# Autodesk Inventor assembly: HALF GANTRY ASSEMBLY
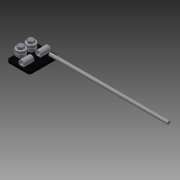
[picture p0: Inventor's stored thumbnail of the model, 180x180]
Saved by Autodesk Inventor 2013 (Build 170138000, 138)
## iProperties
Created: 2014-03-03
Part Number: HALF GANTRY ASSEMBLY
Document SubType Name: Assembly
Designer: employee
Author: employee
## Documents named in this file (8)
- C:\Users\employee\Desktop\CoreXZ\HALF GANTRY ASSEMBLY.iam
- C:\Users\employee\Desktop\CoreXZ\GANTRY SIDE PLATE.ipt
- C:\Users\employee\Desktop\CoreXZ\LM8UU.ipt
- C:\Users\employee\Desktop\CoreXZ\M8X290 ROD.ipt
- C:\Users\employee\Desktop\CoreXZ\SPACER.ipt
- C:\Users\employee\Desktop\CoreXZ\608.ipt
- C:\Users\employee\Desktop\CoreXZ\M8X40.ipt
- C:\Users\employee\Desktop\CoreXZ\M8 NUT.ipt
## Components (14 placed, 7 different names)
1. GANTRY SIDE PLATE:1 — Insert:1, Insert:2, Insert:3, Insert:4, Insert:5, Insert:12, Insert:13
2. LM8UU:1 — Insert:1
3. LM8UU:2 — Insert:2
4. M8X290 ROD:1 — Insert:3
5. SPACER:1 — Insert:5, Insert:8
6. SPACER:2 — Insert:4, Insert:6
7. 608:1 — Insert:7, Insert:10
8. 608:2 — Insert:6, Insert:7
9. 608:3 — Insert:8, Insert:9
10. 608:4 — Insert:9, Insert:11
11. M8X40:1 — Insert:10
12. M8X40:2 — Insert:11
13. M8 NUT:1 — Insert:12
14. M8 NUT:2 — Insert:13
## Relationships (13: Insert 13)
- Insert:1: GANTRY SIDE PLATE:1 ↔ LM8UU:1
- Insert:2: GANTRY SIDE PLATE:1 ↔ LM8UU:2
- Insert:3: GANTRY SIDE PLATE:1 ↔ M8X290 ROD:1
- Insert:4: GANTRY SIDE PLATE:1 ↔ SPACER:2
- Insert:5: GANTRY SIDE PLATE:1 ↔ SPACER:1
- Insert:6: SPACER:2 ↔ 608:2
- Insert:7: 608:1 ↔ 608:2
- Insert:8: SPACER:1 ↔ 608:3
- Insert:9: 608:3 ↔ 608:4
- Insert:10: 608:1 ↔ M8X40:1
- Insert:11: 608:4 ↔ M8X40:2
- Insert:12 (6.477 mm): GANTRY SIDE PLATE:1 ↔ M8 NUT:1
- Insert:13 (6.477 mm): GANTRY SIDE PLATE:1 ↔ M8 NUT:2
